# Autodesk Inventor assembly: hoops_sml_med_lrg
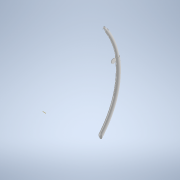
[picture p0: Inventor's stored thumbnail of the model, 180x180]
Saved by Autodesk Inventor 2021 (Build 250183000, 183)
## iProperties
Created: 2021-05-05
Part Number: hoops_sml_med_lrg
Document SubType Name: Assembly
## Documents named in this file (7)
- C:\Users\ocon0143\OneDrive - Flinders\Advn Mech Design Shared\6_Development\2_Design\inventor\hoop_slider\hoops_sml_med_lrg.iam
- C:\Users\ocon0143\OneDrive - Flinders\Advn Mech Design Shared\6_Development\2_Design\inventor\hoop_slider\large_hoop.ipt
- C:\Users\ocon0143\OneDrive - Flinders\Advn Mech Design Shared\6_Development\2_Design\inventor\hoop_slider\medium_hoop.ipt
- C:\Users\ocon0143\OneDrive - Flinders\Advn Mech Design Shared\6_Development\2_Design\inventor\rack_pinion\pinion.ipt
- C:\Users\ocon0143\OneDrive - Flinders\Advn Mech Design Shared\6_Development\2_Design\inventor\hoop_slider\small_hoop.ipt
- C:\Users\ocon0143\OneDrive - Flinders\Advn Mech Design Shared\6_Development\2_Design\inventor\rack_pinion\tooth.ipt
- C:\Users\ocon0143\OneDrive - Flinders\Advn Mech Design Shared\6_Development\2_Design\inventor\rack_pinion\pulley_guide.ipt
## Components (65 placed, 6 different names)
1. large_hoop:1 — Mate:1, Flush:1
2. medium_hoop:1 — Mate:2, Flush:2, Mate:4, Flush:8, Flush:9
3. pinion:1 — Flush:6
4. small_hoop:1 — Mate:3, Flush:7, Flush:10, Mate:5, Flush:11
5. pulley_guide:1 — Flush:10, Mate:5, Flush:11
6. tooth:1 — Mate:4, Flush:8, Flush:9
7. tooth:2
8. tooth:3
9. tooth:4
10. tooth:5
11. tooth:6
12. tooth:7
13. tooth:8
14. tooth:9
15. tooth:10
16. tooth:11
17. tooth:12
18. tooth:13
19. tooth:14
20. tooth:15
21. tooth:16
22. tooth:17
23. tooth:18
24. tooth:19
25. tooth:20
26. tooth:21
27. tooth:22
28. tooth:23
29. tooth:24
30. tooth:25
31. tooth:26
32. tooth:27
33. tooth:28
34. tooth:29
35. tooth:30
36. tooth:31
37. tooth:32
38. tooth:33
39. tooth:34
40. tooth:35
41. tooth:36
42. tooth:37
43. tooth:38
44. tooth:39
45. tooth:40
46. tooth:41
47. tooth:42
48. tooth:43
49. tooth:44
50. tooth:45
51. tooth:46
52. tooth:47
53. tooth:48
54. tooth:49
55. tooth:50
56. tooth:51
57. tooth:52
58. tooth:53
59. tooth:54
60. tooth:55
61. tooth:56
62. tooth:57
63. tooth:58
64. tooth:59
65. tooth:60
## Component patterns: (60 elements, first: tooth:1)
## Relationships (13: Flush 8, Mate 5)
- Mate:1: large_hoop:1
- Mate:2: medium_hoop:1
- Flush:1: large_hoop:1
- Flush:2: medium_hoop:1
- Flush:6: pinion:1
- Mate:3: small_hoop:1
- Flush:7: small_hoop:1
- Mate:4: medium_hoop:1 ↔ tooth:1
- Flush:8: medium_hoop:1 ↔ tooth:1
- Flush:9: medium_hoop:1 ↔ tooth:1
- Flush:10 (4 mm): small_hoop:1 ↔ pulley_guide:1
- Mate:5 (1622 mm): small_hoop:1 ↔ pulley_guide:1
- Flush:11: small_hoop:1 ↔ pulley_guide:1
